# Autodesk Inventor assembly: アーム
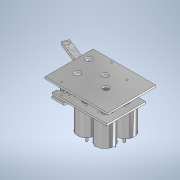
[picture p0: Inventor's stored thumbnail of the model, 180x180]
Saved by Autodesk Inventor 2020.2 (Build 242310000, 310)
## iProperties
Created: 2020-03-16
Part Number: アーム
Document SubType Name: Assembly
Designer: aoyam
Author: aoyam
## Documents named in this file (9)
- C:\Users\aoyam\Desktop\SRDC_local\Inventor\二年機\インナー4層丙\アーム\アーム.iam
- C:\Users\aoyam\Desktop\SRDC_local\Inventor\二年機\インナー4層丙\汎用部品\アーム用初段.iam
- C:\Users\aoyam\Desktop\SRDC_local\Inventor\二年機\インナー4層丙\アーム\モーターマウント.ipt
- C:\Users\aoyam\Desktop\SRDC_local\Inventor\二年機\インナー4層丙\汎用部品\マブチRS380.iam
- C:\Users\aoyam\Desktop\SRDC_local\Inventor\二年機\インナー4層丙\アーム\アーム用2段.iam
- C:\Users\aoyam\Desktop\SRDC_local\Inventor\二年機\インナー4層丙\アーム\アーム用3段.iam
- C:\Users\aoyam\Desktop\SRDC_local\Inventor\二年機\インナー4層丙\アーム\アームフレーム.ipt
- C:\Users\aoyam\Desktop\SRDC_local\Inventor\二年機\インナー4層丙\アーム\駆動軸.ipt
- C:\Users\aoyam\Desktop\SRDC_local\Inventor\二年機\インナー4層丙\アーム\アームフレーム2.ipt
## Components (10 placed, 8 different names)
1. モーターマウント:1 — 挿入:1, メイト:1, 挿入:2, メイト:2, 挿入:3, メイト:3, 挿入:4, メイト:5, メイト:7, メイト:8, メイト:9
2. マブチRS380:1 [sub-assembly] — 挿入:2, メイト:2
3. マブチRS380:2 [sub-assembly] — 挿入:3, メイト:3
4. マブチRS380:3 [sub-assembly] — 挿入:1, メイト:1
5. アーム用初段:1 [sub-assembly] — 挿入:4, メイト:4, 挿入:6
6. アーム用2段:1 [sub-assembly] — メイト:4, メイト:5, メイト:6
7. アーム用3段:1 [sub-assembly] — メイト:6, メイト:10, メイト:11
8. アームフレーム:1 — メイト:7, メイト:8, メイト:9, メイト:10, メイト:11, 挿入:5
9. 駆動軸:1 — 挿入:5, メイト:12
10. アームフレーム2:1 — 挿入:6, メイト:12
## Relationships (18: Mate 12, Insert 6)
- 挿入:1 [Insert]: モーターマウント:1 ↔ マブチRS380:3
- メイト:1 [Mate]: モーターマウント:1 ↔ マブチRS380:3
- 挿入:2 [Insert]: モーターマウント:1 ↔ マブチRS380:1
- メイト:2 [Mate]: モーターマウント:1 ↔ マブチRS380:1
- 挿入:3 [Insert]: モーターマウント:1 ↔ マブチRS380:2
- メイト:3 [Mate]: モーターマウント:1 ↔ マブチRS380:2
- 挿入:4 [Insert] (6 mm): モーターマウント:1 ↔ アーム用初段:1
- メイト:4 [Mate] (0.5 mm): アーム用初段:1 ↔ アーム用2段:1
- メイト:5 [Mate]: モーターマウント:1 ↔ アーム用2段:1
- メイト:6 [Mate] (0.5 mm): アーム用2段:1 ↔ アーム用3段:1
- メイト:7 [Mate]: モーターマウント:1 ↔ アームフレーム:1
- メイト:8 [Mate]: モーターマウント:1 ↔ アームフレーム:1
- メイト:9 [Mate]: モーターマウント:1 ↔ アームフレーム:1
- メイト:10 [Mate]: アーム用3段:1 ↔ アームフレーム:1
- メイト:11 [Mate] (0.5 mm): アーム用3段:1 ↔ アームフレーム:1
- 挿入:5 [Insert] (1 mm): アームフレーム:1 ↔ 駆動軸:1
- 挿入:6 [Insert] (0.5 mm): アーム用初段:1 ↔ アームフレーム2:1
- メイト:12 [Mate]: 駆動軸:1 ↔ アームフレーム2:1
